# Autodesk Inventor assembly: Torso_automi2
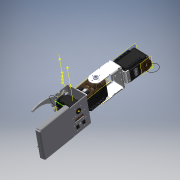
[picture p0: Inventor's stored thumbnail of the model, 180x180]
Saved by Autodesk Inventor 2018 (Build 220112000, 112)
## iProperties
Created: 2018-06-24
Part Number: Torso_automi2
Document SubType Name: Assembly
Designer: ayush
Author: ayush
## Documents named in this file (7)
- C:\Users\Abhay\Desktop\Huro\gripper\Torso_automi2.iam
- C:\Users\Abhay\Desktop\Huro\_18 Summers\Biped\AX-18A.iam
- C:\Users\Abhay\Desktop\Huro\_18 Summers\Biped\AX18_Frame.ipt
- C:\Users\Abhay\Desktop\Huro\_18 Summers\Biped\FP04_Ax18.ipt
- C:\Users\Abhay\Desktop\Huro\_18 Summers\Biped\BPF-BU.ipt
- C:\Users\Abhay\Desktop\Huro\_18 Summers\Biped\BPF-WA.ipt
- C:\Users\Abhay\Desktop\Huro\gripper\Assembly1.iam
## Components (10 placed, 6 different names)
1. AX-18A:5 [sub-assembly] — Rotational:8, Mate:8, Rigid:23, Rotational:23
2. AX18_Frame:4 — Rotational:8, Mate:8, Rotational:11, Mate:11
3. FP04_Ax18:1 — Rotational:11, Mate:11, Rotational:12
4. AX-18A:7 [sub-assembly] — Rotational:12, Rotational:15, Mate:13, Rigid:24, Rotational:24
5. AX18_Frame:6 — Rotational:15, Mate:13, Rotational:28, Mate:18
6. BPF-BU:3 — Rigid:23
7. BPF-BU:4 — Rigid:24
8. BPF-WA:3 — Rotational:24
9. BPF-WA:4 — Rotational:23
10. Assembly1:1 [sub-assembly] — Rotational:28, Mate:18
## Relationships (13: RevoluteJoint 7, Mate 4, WeldJoint 2)
- Rotational:8 [RevoluteJoint]: AX-18A:5 ↔ AX18_Frame:4
- Mate:8: AX-18A:5 ↔ AX18_Frame:4
- Rotational:11 [RevoluteJoint]: AX18_Frame:4 ↔ FP04_Ax18:1
- Mate:11: AX18_Frame:4 ↔ FP04_Ax18:1
- Rotational:12 [RevoluteJoint] (-1 mm): FP04_Ax18:1 ↔ AX-18A:7
- Rotational:15 [RevoluteJoint] (-1 mm): AX-18A:7 ↔ AX18_Frame:6
- Mate:13: AX-18A:7 ↔ AX18_Frame:6
- Rigid:23 [WeldJoint]: AX-18A:5 ↔ BPF-BU:3
- Rotational:23 [RevoluteJoint]: AX-18A:5 ↔ BPF-WA:4
- Rigid:24 [WeldJoint]: AX-18A:7 ↔ BPF-BU:4
- Rotational:24 [RevoluteJoint]: AX-18A:7 ↔ BPF-WA:3
- Rotational:28 [RevoluteJoint]: AX18_Frame:6 ↔ Assembly1:1
- Mate:18: AX18_Frame:6 ↔ Assembly1:1
